# Autodesk Inventor assembly: theperfectone
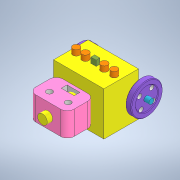
[picture p0: Inventor's stored thumbnail of the model, 180x180]
Saved by Autodesk Inventor 2021 (Build 250183000, 183)
## iProperties
Created: 2021-07-26
Part Number: theperfectone
Document SubType Name: Assembly
Designer: Dell
Author: Dell
## Documents named in this file (5)
- C:\Users\Dell\Desktop\theperfectone.iam
- C:\Users\Dell\Desktop\newcylinder1.ipt
- C:\Users\Dell\Desktop\finalface4.ipt
- C:\Users\Dell\Desktop\thesmallest.ipt
- C:\Users\Dell\Desktop\1.4cylinder.ipt
## Components (5 placed, 4 different names)
1. newcylinder1:1 — Mate:1, Rotational:1
2. finalface4:1 — Mate:1
3. 1.4cylinder:1 — Rotational:1, Rigid:1, Rigid:2
4. thesmallest:1 — Rigid:2
5. thesmallest:2 — Rigid:1
## Relationships (4: WeldJoint 2, Mate 1, RevoluteJoint 1)
- Mate:1: newcylinder1:1 ↔ finalface4:1
- Rotational:1 [RevoluteJoint]: newcylinder1:1 ↔ 1.4cylinder:1
- Rigid:1 [WeldJoint] (-4.7625 mm): 1.4cylinder:1 ↔ thesmallest:2
- Rigid:2 [WeldJoint] (4.7625 mm): 1.4cylinder:1 ↔ thesmallest:1
